# Autodesk Inventor assembly: Roller
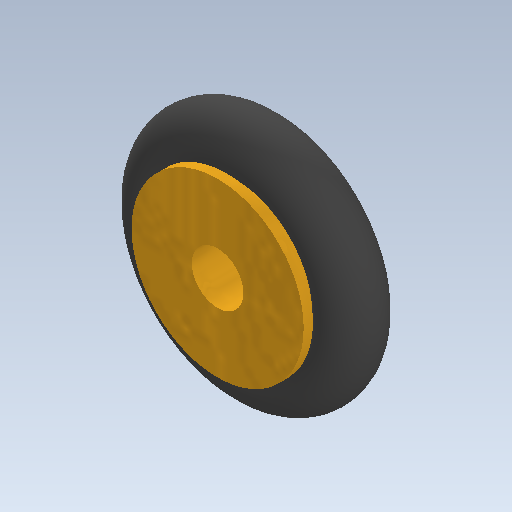
[picture p0: Inventor's stored thumbnail of the model, 512x512]
Saved by Autodesk Inventor 2020 (Build 240168000, 168)
## iProperties
Created: 2021-05-01
Part Number: Roller
Document SubType Name: Assembly
Designer: Acer
Author: Acer
## Documents named in this file (3)
- G:\Meu Drive\RobôCIn\Mecânica\SSL\2021\Inventor\first_floor\Wheel\Roller.iam
- G:\Meu Drive\RobôCIn\Mecânica\SSL\2021\Inventor\first_floor\Wheel\Roller.ipt
- G:\Meu Drive\RobôCIn\Mecânica\SSL\2021\Inventor\first_floor\Wheel\RollerTire.ipt
## Components (2 placed, 2 different names)
1. Roller:1 — Rigid:1
2. RollerTire:1 — Rigid:1
## Relationships (1: WeldJoint 1)
- Rigid:1 [WeldJoint]: Roller:1 ↔ RollerTire:1
